# Autodesk Inventor assembly: poleStand
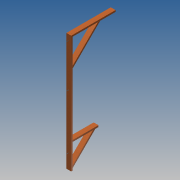
[picture p0: Inventor's stored thumbnail of the model, 180x180]
Saved by Autodesk Inventor 2014 SP1 (Build 180222100, 222)
## iProperties
Created: 2013-12-02
Part Number: poleStand
Document SubType Name: Assembly
Designer: Dave
Author: Dave
## Documents named in this file (8)
- C:\Users\Dave\Desktop\hera-cad\support\poleStandVertAssy.iam
- C:\Users\Dave\Desktop\hera-cad\support\poleStandVert.ipt
- C:\Users\Dave\Desktop\hera-cad\support\poleStandHoriz1.ipt
- C:\Users\Dave\Desktop\hera-cad\support\poleStand45.ipt
- C:\Users\Dave\Desktop\hera-cad\support\poleScreenHldHoriz.ipt
- C:\Users\Dave\Desktop\hera-cad\support\poleScreenHld45.ipt
- C:\Users\Dave\Desktop\hera-cad\smallParts\washer_3-8.ipt
- C:\Users\Dave\Desktop\hera-cad\smallParts\lagBolt_3-8.ipt
## Components (11 placed, 7 different names)
1. poleStandVert:1 — Insert:1, Mate:1, Flush:4, Flush:5, Mate:3, Insert:3, Insert:4, Insert:5, Flush:7, Flush:8, Mate:4
2. poleStand45:1 — Flush:8, Mate:4, Mate:5
3. poleStandHoriz1:1 — Insert:1, Flush:7, Mate:5
4. poleScreenHldHoriz:1 — Mate:1, Flush:4, Flush:5, Mate:2, Flush:6
5. poleScreenHld45:1 — Mate:2, Mate:3, Flush:6
6. washer_3-8:1 — Insert:3, Insert:6
7. washer_3-8:2 — Insert:4, Insert:7
8. washer_3-8:3 — Insert:5, Insert:8
9. lagBolt_3-8:1 — Insert:8
10. lagBolt_3-8:2 — Insert:7
11. lagBolt_3-8:3 — Insert:6
## Relationships (17: Insert 7, Mate 5, Flush 5)
- Insert:1: poleStandVert:1 ↔ poleStandHoriz1:1
- Mate:1: poleStandVert:1 ↔ poleScreenHldHoriz:1
- Flush:4: poleStandVert:1 ↔ poleScreenHldHoriz:1
- Flush:5: poleStandVert:1 ↔ poleScreenHldHoriz:1
- Mate:2: poleScreenHldHoriz:1 ↔ poleScreenHld45:1
- Mate:3: poleStandVert:1 ↔ poleScreenHld45:1
- Flush:6 (-1.651 mm): poleScreenHldHoriz:1 ↔ poleScreenHld45:1
- Insert:3: poleStandVert:1 ↔ washer_3-8:1
- Insert:4: poleStandVert:1 ↔ washer_3-8:2
- Insert:5: poleStandVert:1 ↔ washer_3-8:3
- Insert:6: washer_3-8:1 ↔ lagBolt_3-8:3
- Insert:7: washer_3-8:2 ↔ lagBolt_3-8:2
- Insert:8: washer_3-8:3 ↔ lagBolt_3-8:1
- Flush:7: poleStandVert:1 ↔ poleStandHoriz1:1
- Flush:8: poleStandVert:1 ↔ poleStand45:1
- Mate:4: poleStandVert:1 ↔ poleStand45:1
- Mate:5: poleStand45:1 ↔ poleStandHoriz1:1
